# Autodesk Inventor assembly: climb
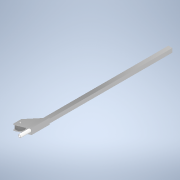
[picture p0: Inventor's stored thumbnail of the model, 180x180]
Saved by Autodesk Inventor 2020 (Build 240168000, 168)
## iProperties
Created: 2020-01-25
Part Number: climb
Document SubType Name: Assembly
Designer: 1jyng
Author: 1jyng
## Documents named in this file (7)
- J:\Writable\Iron Riders\Robot 2020\Climber\climb.iam
- J:\Writable\Iron Riders\Robot 2020\Climber\climb 1x1.ipt
- J:\Writable\Iron Riders\Robot 2020\Climber\climb pvc.ipt
- J:\Writable\Iron Riders\Robot 2020\Climber\pulley holder.ipt
- J:\Writable\Iron Riders\Robot 2020\Climber\bottom piece pvc.ipt
- J:\Writable\Iron Riders\Robot 2020\Climber\pulley rod.ipt
- J:\Writable\Iron Riders\Robot 2020\Climber\pulley.ipt
## Components (7 placed, 6 different names)
1. climb 1x1:1 — Mate:1, Flush:3, Mate:2, Flush:4, Mate:3, Mate:4, Flush:5, Mate:5, Mate:6, Flush:6
2. climb pvc:1 — Flush:5, Mate:5, Mate:6, Mate:7
3. pulley holder:1 — Mate:1, Flush:3, Mate:3, Mate:8, Mate:9, Mate:10, Mate:13, Mate:14, Mate:15
4. pulley holder:2 — Mate:2, Flush:4, Mate:4, Mate:11
5. bottom piece pvc:1 — Mate:7, Flush:6
6. pulley rod:1 — Mate:8, Mate:9, Mate:10, Mate:11, Mate:12, Mate:14, Mate:15
7. pulley:1 — Mate:12, Mate:13
## Relationships (19: Mate 15, Flush 4)
- Mate:1: climb 1x1:1 ↔ pulley holder:1
- Flush:3: climb 1x1:1 ↔ pulley holder:1
- Mate:2: climb 1x1:1 ↔ pulley holder:2
- Flush:4: climb 1x1:1 ↔ pulley holder:2
- Mate:3: climb 1x1:1 ↔ pulley holder:1
- Mate:4: climb 1x1:1 ↔ pulley holder:2
- Flush:5 (12.7 mm): climb 1x1:1 ↔ climb pvc:1
- Mate:5 (9.525 mm): climb 1x1:1 ↔ climb pvc:1
- Mate:6 (9.525 mm): climb 1x1:1 ↔ climb pvc:1
- Mate:7: climb pvc:1 ↔ bottom piece pvc:1
- Flush:6: climb 1x1:1 ↔ bottom piece pvc:1
- Mate:8: pulley holder:1 ↔ pulley rod:1
- Mate:9: pulley holder:1 ↔ pulley rod:1
- Mate:10: pulley holder:1 ↔ pulley rod:1
- Mate:11: pulley holder:2 ↔ pulley rod:1
- Mate:12: pulley rod:1 ↔ pulley:1
- Mate:13 (6.35 mm): pulley holder:1 ↔ pulley:1
- Mate:14: pulley holder:1 ↔ pulley rod:1
- Mate:15: pulley holder:1 ↔ pulley rod:1
